# Autodesk Inventor assembly: 102.001.01_Vereinzelung_Gesamtbaugruppe
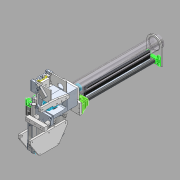
[picture p0: Inventor's stored thumbnail of the model, 180x180]
Saved by Autodesk Inventor 2021 (Build 250183000, 183)
## iProperties
Created: 2021-11-14
Part Number: 102.001.01_Vereinzelung_Gesamtbaugruppe
Document SubType Name: Assembly
Designer: Oliver Ungerer
Sending System: Creo  TM  4.0
KODE_ZEICHNUNGSNUMMER: TFVEM_100M
BENENNUNG: Vereinzelungsmechanismus
BEARBEITER_NAME: Ungerer O.
MASSE: 6.946813
PDMREV: 0.0+
PDMRL: Entwicklung
PROI_REVISION: 0
PROI_VERSION: 0+
PROI_RELEASE: Entwicklung
PTC_MODIFIED: True
PROI_CREATED_BY: Kantioler_adm
PROI_CREATED_ON: 07.03.2008 12:11:19
PROI_LOCATION: Root-Ordner/Pro_stds/Start_Files
MATERIALART: -
EINHEIT: ST
HERSTELLER_PREIS: 0.0
PRUEFER_NAME: Uo
PTC_ORGANIZATION_ID: Durst
PTC_WM_REVISION: 0
PTC_WM_ITERATION: 0
PTC_WM_VERSION: 0.0
PTC_WM_LIFECYCLE_STATE: Entwicklung
PTC_WM_LIFECYCLE: 02 Durst
PTC_WM_CREATED_BY: Oliver Ungerer (oungerer: Durst)
PTC_WM_CREATED_ON: 01.08.21
PTC_WM_MODIFIED_BY: Oliver Ungerer (oungerer: Durst)
PTC_WM_MODIFIED_ON: 01.08.21
AEND_INDEX: 0
VERSION: 0
STATUS: 0.0
Author: Oliver Ungerer
## Documents named in this file (25)
- E:\Dokumente\MCI-Mechatronik\Master\Semester_3\Projekt2_CAD\102_Vereinzelung\102.001.01_Vereinzelung_Gesamtbaugruppe.iam
- E:\Dokumente\MCI-Mechatronik\Master\Semester_3\Projekt2_CAD\102_Vereinzelung\TFVEM_1000.ipt
- E:\Dokumente\MCI-Mechatronik\Master\Semester_3\Projekt2_CAD\102_Vereinzelung\TFVEM_1001.ipt
- E:\Dokumente\MCI-Mechatronik\Master\Semester_3\Projekt2_CAD\102_Vereinzelung\202.001.01_Schieberbetaetigung.iam
- E:\Dokumente\MCI-Mechatronik\Master\Semester_3\Projekt2_CAD\102_Vereinzelung\TFVEM_1002.ipt
- E:\Dokumente\MCI-Mechatronik\Master\Semester_3\Projekt2_CAD\102_Vereinzelung\TFVEM_1003.ipt
- E:\Dokumente\MCI-Mechatronik\Master\Semester_3\Projekt2_CAD\102_Vereinzelung\0001_FLASCHE.ipt
- E:\Dokumente\MCI-Mechatronik\Master\Semester_3\Projekt2_CAD\102_Vereinzelung\TFVEM_1007.ipt
- E:\Dokumente\MCI-Mechatronik\Master\Semester_3\Projekt2_CAD\102_Vereinzelung\TFVEM_1010.ipt
- E:\Dokumente\MCI-Mechatronik\Master\Semester_3\Projekt2_CAD\102_Vereinzelung\_BALLUFF_BIS_M-305-ANTENNE.ipt
- E:\Dokumente\MCI-Mechatronik\Master\Semester_3\Projekt2_CAD\102_Vereinzelung\TFVEM_1011.ipt
- E:\Dokumente\MCI-Mechatronik\Master\Semester_3\Projekt2_CAD\102_Vereinzelung\BALLUFF_BCS_M18BBN1-PSC80D-EP02.ipt
- E:\Dokumente\MCI-Mechatronik\Master\Semester_3\Projekt2_CAD\102_Vereinzelung\TFVEM_1018.ipt
- E:\Dokumente\MCI-Mechatronik\Master\Semester_3\Projekt2_CAD\102_Vereinzelung\TFVEM_1015.ipt
- E:\Dokumente\MCI-Mechatronik\Master\Semester_3\Projekt2_CAD\102_Vereinzelung\TFVEM_1016.ipt
- E:\Dokumente\MCI-Mechatronik\Master\Semester_3\Projekt2_CAD\102_Vereinzelung\TFVEM_1017.ipt
- E:\Dokumente\MCI-Mechatronik\Master\Semester_3\Projekt2_CAD\102_Vereinzelung\TFVEM_1020.ipt
- E:\Dokumente\MCI-Mechatronik\Master\Semester_3\Projekt2_CAD\102_Vereinzelung\TFVEM_1021.ipt
- E:\Dokumente\MCI-Mechatronik\Master\Semester_3\Projekt2_CAD\102_Vereinzelung\TFVEM_1022.ipt
- E:\Dokumente\MCI-Mechatronik\Master\Semester_3\Projekt2_CAD\102_Vereinzelung\TFVEM_1023.ipt
- E:\Dokumente\MCI-Mechatronik\Master\Semester_3\Projekt2_CAD\102_Vereinzelung\TFVEM_1024.ipt
- E:\Dokumente\MCI-Mechatronik\Master\Semester_3\Projekt2_CAD\102_Vereinzelung\TFVEM_1025.ipt
- E:\Dokumente\MCI-Mechatronik\Master\Semester_3\Projekt2_CAD\102_Vereinzelung\102.001.02_Anbindung_Vereinzelung.ipt
- E:\Dokumente\MCI-Mechatronik\Master\Semester_3\Projekt2_CAD\102_Vereinzelung\102.001.03_Justage_Vereinzelung.ipt
- E:\Dokumente\MCI-Mechatronik\Master\Semester_3\Projekt2_CAD\102_Vereinzelung\102.003.01_Anbindung_Vereinzelung.ipt
## Components (30 placed, 22 different names)
1. TFVEM_1000 — Passend:15, Passend:16, Passend:17, Passend:18, Passend:21, Passend:25, Passend:27, Passend:43, Passend:47, Passend:48, Passend:49
2. TFVEM_1001 — Passend:13, Fluchtend:1, Passend:14, Fluchtend:2, Passend:15, Passend:16, Passend:17, Fluchtend:3, Passend:26, Fluchtend:4, Fluchtend:5, Passend:44, Passend:45, Fluchtend:11
3. 202.001.01_Schieberbetaetigung [sub-assembly] — Passend:2, Passend:3, Passend:4, Passend:52, Passend:53, Passend:54
4. TFVEM_1002 — Passend:14, Fluchtend:2, Passend:21, Passend:22, Passend:23, Passend:24, Passend:30, Passend:31, Passend:32
5. TFVEM_1003 — Passend:6, Passend:7, Passend:8, Passend:10, Passend:12, Passend:43, Passend:44, Passend:45
6. 0001_FLASCHE — Passend:18, Fluchtend:3, Passend:19, Passend:20
7. 0001_FLASCHE:1 — Passend:19, Passend:20
8. TFVEM_1007 — Passend:40, Passend:41, Passend:42
9. TFVEM_1010 — Passend:2, Passend:3, Passend:4, Passend:47, Passend:48, Passend:49
10. _BALLUFF_BIS_M-305-ANTENNE — Passend:52, Passend:53, Passend:54
11. TFVEM_1011 — Passend:22, Passend:23, Passend:24, Passend:28
12. TFVEM_1011:1 — Passend:25, Passend:26, Passend:27, Passend:29
13. BALLUFF_BCS_M18BBN1-PSC80D-EP02 — Passend:28, Fluchtend:4
14. BALLUFF_BCS_M18BBN1-PSC80D-EP02:1 — Passend:29, Fluchtend:5
15. TFVEM_1018
16. TFVEM_1015
17. TFVEM_1015:1
18. TFVEM_1016
19. TFVEM_1017
20. TFVEM_1020 — Passend:30, Passend:31, Passend:32, Passend:33, Fluchtend:6, Fluchtend:7, Fluchtend:8, Fluchtend:9, Passend:34, Passend:40
21. TFVEM_1021 — Passend:33, Fluchtend:6, Fluchtend:7, Passend:41, Passend:46, Fluchtend:10
22. TFVEM_1022 — Passend:35, Passend:36, Winkel:1, Passend:37, Passend:38, Winkel:2
23. TFVEM_1023 — Fluchtend:8, Fluchtend:9, Passend:34, Passend:35, Passend:36, Winkel:1
24. TFVEM_1024 — Passend:37, Passend:38, Winkel:2, Passend:39, Winkel:3
25. TFVEM_1025 — Passend:39, Passend:42, Winkel:3
26. 102.001.02_Anbindung_Vereinzelung:1 — Passend:6, Passend:7, Passend:8, Passend:9, Passend:11
27. 102.001.02_Anbindung_Vereinzelung:2 — Passend:9, Passend:10
28. 102.001.02_Anbindung_Vereinzelung:3 — Passend:11, Passend:12
29. 102.001.02_Anbindung_Vereinzelung:4 — Passend:13, Fluchtend:1, Fluchtend:11
30. BALLUFF_BCS_M18BBN1-PSC80D-EP02:3 — Passend:46, Fluchtend:10
## Relationships (64: Mate 50, Flush 11, Angle 3)
- Passend:2 [Mate]: 202.001.01_Schieberbetaetigung ↔ TFVEM_1010
- Passend:3 [Mate]: 202.001.01_Schieberbetaetigung ↔ TFVEM_1010
- Passend:4 [Mate]: 202.001.01_Schieberbetaetigung ↔ TFVEM_1010
- Passend:6 [Mate]: TFVEM_1003 ↔ 102.001.02_Anbindung_Vereinzelung:1
- Passend:7 [Mate]: TFVEM_1003 ↔ 102.001.02_Anbindung_Vereinzelung:1
- Passend:8 [Mate] (25 mm): TFVEM_1003 ↔ 102.001.02_Anbindung_Vereinzelung:1
- Passend:9 [Mate]: 102.001.02_Anbindung_Vereinzelung:1 ↔ 102.001.02_Anbindung_Vereinzelung:2
- Passend:10 [Mate]: TFVEM_1003 ↔ 102.001.02_Anbindung_Vereinzelung:2
- Passend:11 [Mate]: 102.001.02_Anbindung_Vereinzelung:1 ↔ 102.001.02_Anbindung_Vereinzelung:3
- Passend:12 [Mate]: TFVEM_1003 ↔ 102.001.02_Anbindung_Vereinzelung:3
- Passend:13 [Mate]: TFVEM_1001 ↔ 102.001.02_Anbindung_Vereinzelung:4
- Fluchtend:1 [Flush]: TFVEM_1001 ↔ 102.001.02_Anbindung_Vereinzelung:4
- Passend:14 [Mate]: TFVEM_1001 ↔ TFVEM_1002
- Fluchtend:2 [Flush]: TFVEM_1001 ↔ TFVEM_1002
- Passend:15 [Mate]: TFVEM_1000 ↔ TFVEM_1001
- Passend:16 [Mate]: TFVEM_1000 ↔ TFVEM_1001
- Passend:17 [Mate]: TFVEM_1000 ↔ TFVEM_1001
- Passend:18 [Mate]: TFVEM_1000 ↔ 0001_FLASCHE
- Fluchtend:3 [Flush]: TFVEM_1001 ↔ 0001_FLASCHE
- Passend:19 [Mate]: 0001_FLASCHE ↔ 0001_FLASCHE:1
- Passend:20 [Mate]: 0001_FLASCHE ↔ 0001_FLASCHE:1
- Passend:21 [Mate]: TFVEM_1000 ↔ TFVEM_1002
- Passend:22 [Mate]: TFVEM_1002 ↔ TFVEM_1011
- Passend:23 [Mate]: TFVEM_1002 ↔ TFVEM_1011
- Passend:24 [Mate]: TFVEM_1002 ↔ TFVEM_1011
- Passend:25 [Mate]: TFVEM_1000 ↔ TFVEM_1011:1
- Passend:26 [Mate]: TFVEM_1001 ↔ TFVEM_1011:1
- Passend:27 [Mate]: TFVEM_1000 ↔ TFVEM_1011:1
- Passend:28 [Mate]: TFVEM_1011 ↔ BALLUFF_BCS_M18BBN1-PSC80D-EP02
- Fluchtend:4 [Flush]: TFVEM_1001 ↔ BALLUFF_BCS_M18BBN1-PSC80D-EP02
- Passend:29 [Mate]: TFVEM_1011:1 ↔ BALLUFF_BCS_M18BBN1-PSC80D-EP02:1
- Fluchtend:5 [Flush]: TFVEM_1001 ↔ BALLUFF_BCS_M18BBN1-PSC80D-EP02:1
- Passend:30 [Mate]: TFVEM_1002 ↔ TFVEM_1020
- Passend:31 [Mate]: TFVEM_1002 ↔ TFVEM_1020
- Passend:32 [Mate]: TFVEM_1002 ↔ TFVEM_1020
- Passend:33 [Mate]: TFVEM_1020 ↔ TFVEM_1021
- Fluchtend:6 [Flush]: TFVEM_1020 ↔ TFVEM_1021
- Fluchtend:7 [Flush]: TFVEM_1020 ↔ TFVEM_1021
- Fluchtend:8 [Flush]: TFVEM_1020 ↔ TFVEM_1023
- Fluchtend:9 [Flush]: TFVEM_1020 ↔ TFVEM_1023
- Passend:34 [Mate]: TFVEM_1020 ↔ TFVEM_1023
- Passend:35 [Mate]: TFVEM_1022 ↔ TFVEM_1023
- Passend:36 [Mate]: TFVEM_1022 ↔ TFVEM_1023
- Winkel:1 [Angle] (180 deg): TFVEM_1022 ↔ TFVEM_1023
- Passend:37 [Mate]: TFVEM_1022 ↔ TFVEM_1024
- Passend:38 [Mate]: TFVEM_1022 ↔ TFVEM_1024
- Winkel:2 [Angle] (180 deg): TFVEM_1022 ↔ TFVEM_1024
- Passend:39 [Mate]: TFVEM_1024 ↔ TFVEM_1025
- Passend:40 [Mate]: TFVEM_1007 ↔ TFVEM_1020
- Passend:41 [Mate]: TFVEM_1007 ↔ TFVEM_1021
- Passend:42 [Mate]: TFVEM_1007 ↔ TFVEM_1025
- Winkel:3 [Angle] (0 deg): TFVEM_1024 ↔ TFVEM_1025
- Passend:43 [Mate]: TFVEM_1000 ↔ TFVEM_1003
- Passend:44 [Mate]: TFVEM_1001 ↔ TFVEM_1003
- Passend:45 [Mate]: TFVEM_1001 ↔ TFVEM_1003
- Passend:46 [Mate]: TFVEM_1021 ↔ BALLUFF_BCS_M18BBN1-PSC80D-EP02:3
- Fluchtend:10 [Flush] (10 mm): TFVEM_1021 ↔ BALLUFF_BCS_M18BBN1-PSC80D-EP02:3
- Passend:47 [Mate]: TFVEM_1000 ↔ TFVEM_1010
- Passend:48 [Mate]: TFVEM_1000 ↔ TFVEM_1010
- Passend:49 [Mate]: TFVEM_1000 ↔ TFVEM_1010
- Passend:52 [Mate]: 202.001.01_Schieberbetaetigung ↔ _BALLUFF_BIS_M-305-ANTENNE
- Passend:53 [Mate]: 202.001.01_Schieberbetaetigung ↔ _BALLUFF_BIS_M-305-ANTENNE
- Passend:54 [Mate]: 202.001.01_Schieberbetaetigung ↔ _BALLUFF_BIS_M-305-ANTENNE
- Fluchtend:11 [Flush]: TFVEM_1001 ↔ 102.001.02_Anbindung_Vereinzelung:4
